# Autodesk Inventor assembly: Design 2
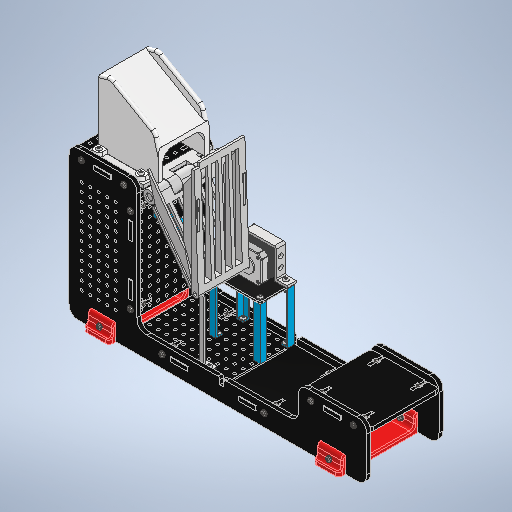
[picture p0: Inventor's stored thumbnail of the model, 512x512]
Saved by Autodesk Inventor 2025.1 (Build 291241020, 241B)
## iProperties
Created: 2024-10-25
Part Number: Design 2
Document SubType Name: Assembly
Designer: aly_g
Author: aly_g
## Documents named in this file (18)
- C:\Users\aly_g\Downloads\School\Eng Design\P1\CAD Model\Finalized Design.iam
- C:\Users\aly_g\Downloads\School\Eng Design\P1\CAD Model\Platform Assembly\1. Platform\Mechanism Platform.iam
- C:\Users\aly_g\Downloads\School\Eng Design\P1\CAD Model\Rotary Actuator Mount.ipt
- C:\Users\aly_g\Downloads\School\Eng Design\P1\CAD Model\Rotary Actuator Assembly\4. Rotary Actuator\Stepper Motor NEMA 17.iam
- C:\Users\aly_g\Downloads\School\Eng Design\P1\CAD Model\Rotary Actuator Platform Design 2.ipt
- C:\Users\aly_g\Downloads\School\Eng Design\P1\CAD Model\Hinge Assembly.iam
- C:\Users\aly_g\Downloads\School\Eng Design\P1\CAD Model\Top Ramp.ipt
- C:\Users\aly_g\Downloads\School\Eng Design\P1\CAD Model\Hinge Siderail 1.ipt
- C:\Users\aly_g\Downloads\School\Eng Design\P1\CAD Model\Hinge Siderail 2.ipt
- C:\Users\aly_g\Downloads\School\Eng Design\P1\CAD Model\Legs.ipt
- C:\Users\aly_g\Downloads\School\Eng Design\P1\CAD Model\Ramp 2.ipt
- C:\Users\aly_g\Downloads\School\Eng Design\P1\CAD Model\Moving Ramp Inside Rail.ipt
- C:\Users\aly_g\Downloads\School\Eng Design\P1\CAD Model\Hinge Holder.ipt
- C:\Users\aly_g\Downloads\School\Eng Design\P1\CAD Model\Moving Ramp Holder.ipt.iam
- C:\Users\aly_g\Downloads\School\Eng Design\P1\CAD Model\2. Plate Fasteners\2. Plate Fasteners\M4 x 20mm Machine Screw.ipt
- C:\Users\aly_g\Downloads\School\Eng Design\P1\CAD Model\2. Plate Fasteners\2. Plate Fasteners\M4 x 16mm Machine Screw.ipt
- C:\Users\aly_g\Downloads\School\Eng Design\P1\CAD Model\2. Plate Fasteners\2. Plate Fasteners\M4 Nut.ipt
- Moving Ramp Holder.ipt
## Components (47 placed, 16 different names)
1. Mechanism Platform:1 [sub-assembly] — Insert:1, Insert:2, Insert:5, Angle:1, Angle:2, Insert:11, Insert:12, Insert:13, Insert:17, Insert:18, Insert:19, Angle:5, Insert:39, Insert:40, Insert:41, Insert:42, Insert:43, Insert:44, Insert:45, Insert:46, Insert:47, Insert:48, Insert:49
2. Hinge Holder:1 — Insert:19, Angle:5, Insert:34
3. Moving Ramp Rail:1 — Mate:8, Mate:11, Mate:13
4. Hinge Siderail 1:1 — Mate:1, Mate:2, Mate:15
5. Hinge Siderail 2:1 — Mate:3, Mate:4, Mate:14
6. Ramp 1:1 — Mate:7, Insert:16, Mate:8, Mate:9, Mate:10, Mate:11, Mate:12, Mate:13
7. Hinge Assembly:1 [sub-assembly] — Insert:1, Insert:2, Mate:1, Mate:2, Mate:3, Mate:4, Insert:3, Insert:4, Mate:14, Mate:15
8. Top Ramp:1 — Insert:3, Insert:4, Insert:20, Insert:21, Insert:22, Insert:23
9. Legs:1 — Insert:5, Angle:2, Insert:9, Insert:28, Insert:38
10. Legs:2 — Insert:8, Angle:3, Insert:12, Insert:27, Insert:35
11. Legs:3 — Angle:1, Insert:10, Insert:11, Insert:29, Insert:36
12. Legs:4 — Insert:7, Angle:4, Insert:13, Insert:26, Insert:37
13. Rotary Actuator Platform Design 2:2 — Insert:7, Insert:8, Angle:3, Angle:4, Insert:9, Insert:10, Mate:5, Flush:3, Insert:14, Insert:15, Insert:25, Insert:31
14. Rotary Actuator Mount:1 — Insert:14, Insert:15, Mate:6, Insert:24, Insert:30
15. Stepper Motor NEMA 17:1 [sub-assembly] — Mate:5, Flush:3, Mate:6, Mate:7, Insert:16
16. Moving Ramp Holder.ipt:1 [sub-assembly] — Insert:17, Insert:18, Insert:32, Insert:33
17. Moving Ramp Rail:2 — Mate:9, Mate:10, Mate:12
18. M4 x 20mm Machine Screw:1 — Insert:20
19. M4 x 20mm Machine Screw:2 — Insert:21
20. M4 x 20mm Machine Screw:3 — Insert:23
21. M4 x 20mm Machine Screw:4 — Insert:22
22. M4 x 16mm Machine Screw:1 — Insert:26
23. M4 x 16mm Machine Screw:2 — Insert:25
24. M4 x 16mm Machine Screw:3 — Insert:24
25. M4 x 16mm Machine Screw:4 — Insert:32
26. M4 x 16mm Machine Screw:5 — Insert:31
27. M4 x 16mm Machine Screw:6 — Insert:28
28. M4 x 16mm Machine Screw:7 — Insert:27
29. M4 x 16mm Machine Screw:8 — Insert:29
30. M4 x 16mm Machine Screw:9 — Insert:30
31. M4 x 16mm Machine Screw:10 — Insert:33
32. M4 x 16mm Machine Screw:11 — Insert:34
33. M4 Nut:1 — Insert:36
34. M4 Nut:2 — Insert:35
35. M4 Nut:3 — Insert:38
36. M4 Nut:4 — Insert:42
37. M4 Nut:5 — Insert:37
38. M4 Nut:6 — Insert:40
39. M4 Nut:7 — Insert:41
40. M4 Nut:8 — Insert:39
41. M4 Nut:9 — Insert:43
42. M4 Nut:10 — Insert:44
43. M4 Nut:11 — Insert:45
44. M4 Nut:12 — Insert:49
45. M4 Nut:13 — Insert:48
46. M4 Nut:14 — Insert:47
47. M4 Nut:15 — Insert:46
## Relationships (69: Insert 48, Mate 15, Angle 5, Flush 1)
- Insert:1: Mechanism Platform:1 ↔ Hinge Assembly:1
- Insert:2: Mechanism Platform:1 ↔ Hinge Assembly:1
- Mate:1: Hinge Siderail 1:1 ↔ Hinge Assembly:1
- Mate:2: Hinge Siderail 1:1 ↔ Hinge Assembly:1
- Mate:3: Hinge Siderail 2:1 ↔ Hinge Assembly:1
- Mate:4: Hinge Siderail 2:1 ↔ Hinge Assembly:1
- Insert:3: Hinge Assembly:1 ↔ Top Ramp:1
- Insert:4: Hinge Assembly:1 ↔ Top Ramp:1
- Insert:5: Mechanism Platform:1 ↔ Legs:1
- Angle:1 (0 deg): Mechanism Platform:1 ↔ Legs:3
- Angle:2 (0 deg): Mechanism Platform:1 ↔ Legs:1
- Insert:7: Legs:4 ↔ Rotary Actuator Platform Design 2:2
- Insert:8: Legs:2 ↔ Rotary Actuator Platform Design 2:2
- Angle:3 (0 deg): Legs:2 ↔ Rotary Actuator Platform Design 2:2
- Angle:4 (0 deg): Legs:4 ↔ Rotary Actuator Platform Design 2:2
- Insert:9: Legs:1 ↔ Rotary Actuator Platform Design 2:2
- Insert:10: Legs:3 ↔ Rotary Actuator Platform Design 2:2
- Insert:11: Mechanism Platform:1 ↔ Legs:3
- Insert:12: Mechanism Platform:1 ↔ Legs:2
- Insert:13: Mechanism Platform:1 ↔ Legs:4
- Mate:5: Rotary Actuator Platform Design 2:2 ↔ Stepper Motor NEMA 17:1
- Flush:3: Rotary Actuator Platform Design 2:2 ↔ Stepper Motor NEMA 17:1
- Insert:14: Rotary Actuator Platform Design 2:2 ↔ Rotary Actuator Mount:1
- Insert:15: Rotary Actuator Platform Design 2:2 ↔ Rotary Actuator Mount:1
- Mate:6: Rotary Actuator Mount:1 ↔ Stepper Motor NEMA 17:1
- Mate:7: Ramp 1:1 ↔ Stepper Motor NEMA 17:1
- Insert:16: Ramp 1:1 ↔ Stepper Motor NEMA 17:1
- Mate:8: Moving Ramp Rail:1 ↔ Ramp 1:1
- Mate:9: Ramp 1:1 ↔ Moving Ramp Rail:2
- Mate:10: Ramp 1:1 ↔ Moving Ramp Rail:2
- Mate:11: Moving Ramp Rail:1 ↔ Ramp 1:1
- Mate:12: Ramp 1:1 ↔ Moving Ramp Rail:2
- Mate:13: Moving Ramp Rail:1 ↔ Ramp 1:1
- Insert:17: Mechanism Platform:1 ↔ Moving Ramp Holder.ipt:1
- Insert:18: Mechanism Platform:1 ↔ Moving Ramp Holder.ipt:1
- Insert:19: Mechanism Platform:1 ↔ Hinge Holder:1
- Mate:14: Hinge Siderail 2:1 ↔ Hinge Assembly:1
- Mate:15: Hinge Siderail 1:1 ↔ Hinge Assembly:1
- Angle:5 (0 deg): Mechanism Platform:1 ↔ Hinge Holder:1
- Insert:20: Top Ramp:1 ↔ M4 x 20mm Machine Screw:1
- Insert:21: Top Ramp:1 ↔ M4 x 20mm Machine Screw:2
- Insert:22: Top Ramp:1 ↔ M4 x 20mm Machine Screw:4
- Insert:23: Top Ramp:1 ↔ M4 x 20mm Machine Screw:3
- Insert:24: Rotary Actuator Mount:1 ↔ M4 x 16mm Machine Screw:3
- Insert:25: Rotary Actuator Platform Design 2:2 ↔ M4 x 16mm Machine Screw:2
- Insert:26: Legs:4 ↔ M4 x 16mm Machine Screw:1
- Insert:27: Legs:2 ↔ M4 x 16mm Machine Screw:7
- Insert:28: Legs:1 ↔ M4 x 16mm Machine Screw:6
- Insert:29: Legs:3 ↔ M4 x 16mm Machine Screw:8
- Insert:30: Rotary Actuator Mount:1 ↔ M4 x 16mm Machine Screw:9
- Insert:31: Rotary Actuator Platform Design 2:2 ↔ M4 x 16mm Machine Screw:5
- Insert:32: Moving Ramp Holder.ipt:1 ↔ M4 x 16mm Machine Screw:4
- Insert:33: Moving Ramp Holder.ipt:1 ↔ M4 x 16mm Machine Screw:10
- Insert:34: Hinge Holder:1 ↔ M4 x 16mm Machine Screw:11
- Insert:35: Legs:2 ↔ M4 Nut:2
- Insert:36: Legs:3 ↔ M4 Nut:1
- Insert:37: Legs:4 ↔ M4 Nut:5
- Insert:38: Legs:1 ↔ M4 Nut:3
- Insert:39: Mechanism Platform:1 ↔ M4 Nut:8
- Insert:40: Mechanism Platform:1 ↔ M4 Nut:6
- Insert:41: Mechanism Platform:1 ↔ M4 Nut:7
- Insert:42: Mechanism Platform:1 ↔ M4 Nut:4
- Insert:43: Mechanism Platform:1 ↔ M4 Nut:9
- Insert:44: Mechanism Platform:1 ↔ M4 Nut:10
- Insert:45: Mechanism Platform:1 ↔ M4 Nut:11
- Insert:46: Mechanism Platform:1 ↔ M4 Nut:15
- Insert:47: Mechanism Platform:1 ↔ M4 Nut:14
- Insert:48: Mechanism Platform:1 ↔ M4 Nut:13
- Insert:49: Mechanism Platform:1 ↔ M4 Nut:12
